# Autodesk Inventor assembly: hip
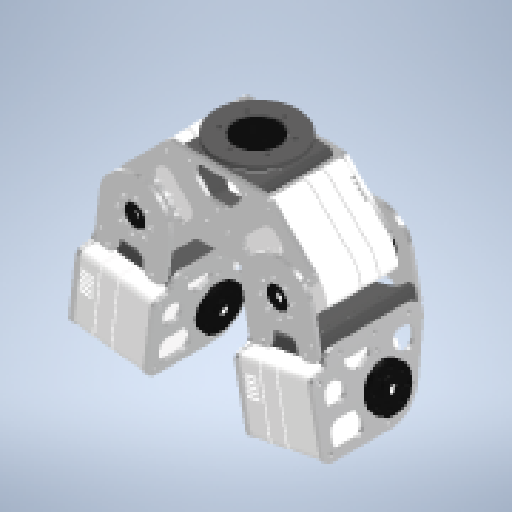
[picture p0: Inventor's stored thumbnail of the model, 512x512]
Saved by Autodesk Inventor 2024.1 (Build 281209000, 209)
## iProperties
Created: 2024-02-12
Part Number: hip
Document SubType Name: Assembly
Designer: hibik
Author: hibik
## Documents named in this file (9)
- C:\Users\hibik\Desktop\ロボメカ\HR\2024.02.11 Rl\02.11 ProtType\hipjoint.iam
- C:\Users\hibik\Desktop\ロボメカ\HR\2024.02.11 Rl\02.11 ProtType\hipjoint.ipt
- C:\Users\hibik\Desktop\ロボメカ\HR\2024.02.11 Rl\KRS3300モータ.ipt
- C:\Users\hibik\Desktop\ロボメカ\HR\2024.02.11 Rl\KRS3300サーボホーン.ipt
- C:\Users\hibik\Desktop\ロボメカ\HR\2024.02.11 Rl\02.11 ProtType\hipjoint_toleg_right.iam
- C:\Users\hibik\Desktop\ロボメカ\HR\2024.02.11 Rl\02.11 ProtType\hipjoint_toleg_left.iam
- C:\Users\hibik\Desktop\ロボメカ\HR\2024.02.11 Rl\02.11 ProtType\hipjoint_middle.ipt
- C:\Users\hibik\Desktop\ロボメカ\HR\2024.02.11 Rl\02.11 ProtType\sholder_joint_c.ipt
- C:\Users\hibik\Desktop\ロボメカ\HR\2024.02.11 Rl\02.11 ProtType\sholder_joint_s.ipt
## Components (18 placed, 8 different names)
1. hipjoint:1 — メイト:3, 角度:1, 角度:2, 挿入:1, 挿入:2, メイト:4, フラッシュ:1, 挿入:14
2. hipjoint:2 — メイト:1, メイト:2, 挿入:3
3. KRS3300モータ:1 — メイト:1, 角度:2, 挿入:2, 挿入:4, 挿入:7
4. KRS3300モータ:2 — メイト:2, メイト:3, 角度:1, 挿入:1, 挿入:3, 挿入:5, 挿入:6
5. KRS3300サーボホーン:1 — 挿入:4, 挿入:9
6. KRS3300サーボホーン:2 — 挿入:5, 挿入:8
7. KRS3300サーボホーン:3 — 挿入:6
8. KRS3300サーボホーン:4 — 挿入:7
9. hipjoint_toleg_right:1 [sub-assembly] — 挿入:9, 挿入:10, 挿入:11
10. hipjoint_toleg_left:1 [sub-assembly] — 挿入:8, 挿入:12, 挿入:13
11. KRS3300サーボホーン:5 — 挿入:10
12. KRS3300サーボホーン:6 — 挿入:11
13. KRS3300サーボホーン:7 — 挿入:12
14. KRS3300サーボホーン:8 — 挿入:13
15. hipjoint_middle:1 — メイト:4, フラッシュ:1, 挿入:14, 挿入:15, 挿入:16
16. KRS3300サーボホーン:9 — 挿入:17, 挿入:18, 挿入:19
17. sholder_joint_c:1 — 挿入:19, 挿入:20
18. sholder_joint_s:1 — 挿入:15, 挿入:16, 挿入:17, 挿入:18, 挿入:20
## Relationships (27: Insert 20, Mate 4, Angle 2, Flush 1)
- メイト:1 [Mate]: hipjoint:2 ↔ KRS3300モータ:1
- メイト:2 [Mate]: hipjoint:2 ↔ KRS3300モータ:2
- メイト:3 [Mate]: hipjoint:1 ↔ KRS3300モータ:2
- 角度:1 [Angle] (0 deg): hipjoint:1 ↔ KRS3300モータ:2
- 角度:2 [Angle] (0 deg): hipjoint:1 ↔ KRS3300モータ:1
- 挿入:1 [Insert]: hipjoint:1 ↔ KRS3300モータ:2
- 挿入:2 [Insert]: hipjoint:1 ↔ KRS3300モータ:1
- 挿入:3 [Insert]: hipjoint:2 ↔ KRS3300モータ:2
- 挿入:4 [Insert] (0.3 mm): KRS3300モータ:1 ↔ KRS3300サーボホーン:1
- 挿入:5 [Insert] (0.3 mm): KRS3300モータ:2 ↔ KRS3300サーボホーン:2
- 挿入:6 [Insert] (0.3 mm): KRS3300モータ:2 ↔ KRS3300サーボホーン:3
- 挿入:7 [Insert] (0.3 mm): KRS3300モータ:1 ↔ KRS3300サーボホーン:4
- 挿入:8 [Insert]: KRS3300サーボホーン:2 ↔ hipjoint_toleg_left:1
- 挿入:9 [Insert]: KRS3300サーボホーン:1 ↔ hipjoint_toleg_right:1
- 挿入:10 [Insert] (0.3 mm): hipjoint_toleg_right:1 ↔ KRS3300サーボホーン:5
- 挿入:11 [Insert] (0.3 mm): hipjoint_toleg_right:1 ↔ KRS3300サーボホーン:6
- 挿入:12 [Insert] (0.3 mm): hipjoint_toleg_left:1 ↔ KRS3300サーボホーン:7
- 挿入:13 [Insert] (0.3 mm): hipjoint_toleg_left:1 ↔ KRS3300サーボホーン:8
- メイト:4 [Mate]: hipjoint:1 ↔ hipjoint_middle:1
- フラッシュ:1 [Flush]: hipjoint:1 ↔ hipjoint_middle:1
- 挿入:14 [Insert]: hipjoint:1 ↔ hipjoint_middle:1
- 挿入:15 [Insert]: hipjoint_middle:1 ↔ sholder_joint_s:1
- 挿入:16 [Insert]: hipjoint_middle:1 ↔ sholder_joint_s:1
- 挿入:17 [Insert]: KRS3300サーボホーン:9 ↔ sholder_joint_s:1
- 挿入:18 [Insert]: KRS3300サーボホーン:9 ↔ sholder_joint_s:1
- 挿入:19 [Insert]: KRS3300サーボホーン:9 ↔ sholder_joint_c:1
- 挿入:20 [Insert]: sholder_joint_c:1 ↔ sholder_joint_s:1
